# Autodesk Inventor assembly: 276-2174
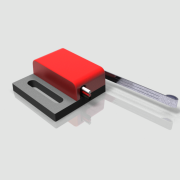
[picture p0: Inventor's stored thumbnail of the model, 180x180]
Saved by Autodesk Inventor 2013 (Build 170138000, 138)
## iProperties
Category: Sensors
Company: Super Sonic Sparks, Team 24
Part Number: 276-2174
Document SubType Name: Assembly
Designer: Jordan Kiesel
Mass: 13.608 g
Surface Area: 67.6196 cm^2
Volume: 5.8262 cm^3
Density: 2.33566 g/cm^3
Catalog Web Link: vexrobotics.com/276-2174.html
Description: Useful as a trigger in a variety of applications.
Vendor: VEX Robotics, Inc.
Translation Standard: STEP AP203
FileName: Limit Switch.iam
PreProcessor: SolidWorks 2006052
PostProcessor: Build: 239, Release: 2011 RTM - Date: Wed 02/17/2010
Sent Units: inch
Uncertainty: 1e-05
Author: Jordan Kiesel
Title: Limit Switch
Comments: Simple limit switch sensor custom built for the VEX Robotics Design System. The switch sends a signal to the Microcontroller when it is triggered. This switch is great for signaling when a robot arm has reached the top or bottom of its motion. ▷ Provide feedback to Microcontroller as events "happen" ▷ Bendable sheet metal switch "arm" is very versatile ▷ Useful as a trigger in a variety of applications ▷ Functionality is pre-programmed in the VEX Microcontroller
## Documents named in this file (5)
- C:\Users\WEBCAST2\Documents\New VEX CAD Parts\Motors & Sensors\Limit Switch.iam
- C:\Users\WEBCAST2\Documents\New VEX CAD Parts\Motors & Sensors\Assembly Parts\Limit Switch\Top.ipt
- C:\Users\WEBCAST2\Documents\New VEX CAD Parts\Motors & Sensors\Assembly Parts\Limit Switch\Microswitch.ipt
- C:\Users\WEBCAST2\Documents\New VEX CAD Parts\Motors & Sensors\Assembly Parts\Limit Switch\Bottom.ipt
- C:\Users\WEBCAST2\Documents\New VEX CAD Parts\Motors & Sensors\Assembly Parts\Sensors\3-Wire Black-Red-White Cable-Cut.ipt
## Components (4 placed, 4 different names)
1. Top:1 — Insert:1, Insert:2, Tangent:1, Tangent:2, Tangent:3
2. Microswitch:1
3. Bottom:1 — Insert:1, Insert:2, Angle:1
4. 3-Wire Black-Red-White Cable-Cut:1 — Tangent:1, Angle:1, Tangent:2, Tangent:3
## Relationships (6: Tangent 3, Insert 2, Angle 1)
- Insert:1: Top:1 ↔ Bottom:1
- Insert:2: Top:1 ↔ Bottom:1
- Tangent:1 (0.889 mm): Top:1 ↔ 3-Wire Black-Red-White Cable-Cut:1
- Angle:1 (0 deg): Bottom:1 ↔ 3-Wire Black-Red-White Cable-Cut:1
- Tangent:2 (4.0894 mm): Top:1 ↔ 3-Wire Black-Red-White Cable-Cut:1
- Tangent:3 (0.221 mm): Top:1 ↔ 3-Wire Black-Red-White Cable-Cut:1
